# Autodesk Inventor assembly: left_gripper_base
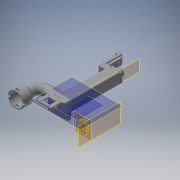
[picture p0: Inventor's stored thumbnail of the model, 180x180]
Saved by Autodesk Inventor 2016 (Build 200138000, 138)
## iProperties
Created: 2016-06-09
Part Number: left_gripper_base
Material: 一般
Document SubType Name: Assembly
Designer: Shun Hasegawa
Author: Shun Hasegawa
## Documents named in this file (4)
- C:\Shun\AmazonPickingChallenge\test3\left\left_gripper_base.iam
- C:\Shun\AmazonPickingChallenge\test3\left\base2.ipt
- C:\Shun\AmazonPickingChallenge\test3\left\tube3.ipt
- C:\Shun\AmazonPickingChallenge\test3\servo.ipt
## Components (3 placed, 3 different names)
1. base2:1 — メイト:1, フラッシュ:1, フラッシュ:2
2. tube3:1 — メイト:1, フラッシュ:1, フラッシュ:2, メイト:2, メイト:3, メイト:4
3. servo:1 — メイト:2, メイト:3, メイト:4
## Relationships (6: Mate 4, Flush 2)
- メイト:1 [Mate]: base2:1 ↔ tube3:1
- フラッシュ:1 [Flush]: base2:1 ↔ tube3:1
- フラッシュ:2 [Flush]: base2:1 ↔ tube3:1
- メイト:2 [Mate]: tube3:1 ↔ servo:1
- メイト:3 [Mate]: tube3:1 ↔ servo:1
- メイト:4 [Mate]: tube3:1 ↔ servo:1
